# Autodesk Inventor assembly: Drivebase
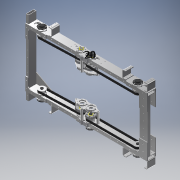
[picture p0: Inventor's stored thumbnail of the model, 180x180]
Saved by Autodesk Inventor 2019.4 (Build 234330000, 330)
## iProperties
Created: 2020-01-05
Part Number: Drivebase
Document SubType Name: Assembly
Designer: Mark
Mass: 11947.6 g
Surface Area: 25724.3 cm^2
Volume: 4557.12 cm^3
Density: 2.62175 g/cm^3
Author: Mark
## Documents named in this file (32)
- C:\Users\Mark\Desktop\7738 Helion Engineering\7738-2020\CAD\Drivebase.iam
- C:\Users\Mark\Desktop\7738 Helion Engineering\7738-2020\CAD\Main Extrusion.ipt
- C:\Users\Mark\Desktop\7738 Helion Engineering\7738-2020\CAD\Back Extrusion.ipt
- C:\Users\Mark\Desktop\7738 Helion Engineering\7738-2020\CAD\Bearing Block Assembly.iam
- C:\Users\Mark\Desktop\7738 Helion Engineering\7738-2020\CAD\Gearbox\Drivebox.iam
- C:\Users\Mark\Desktop\7738 Helion Engineering\7738-2020\CAD\End Extrusion.ipt
- C:\Users\Mark\Desktop\7738 Helion Engineering\7738-2020\CAD\Gearbox\HTD 5M 30 20mm ID Keyed.ipt
- C:\Users\Mark\Desktop\7738 Helion Engineering\7738-2020\CAD\Gearbox\30-30-870-HTD5M.ipt
- C:\Users\Mark\Desktop\7738 Helion Engineering\7738-2020\CAD\Gearbox\30-30-750-HTD5M.ipt
- C:\Users\Mark\Desktop\7738 Helion Engineering\7738-2020\CAD\Frontal Sheet Metal Support.ipt
- C:\Users\Mark\Desktop\7738 Helion Engineering\7738-2020\CAD\Shaft-Secondary.ipt
- C:\Users\Mark\Desktop\7738 Helion Engineering\7738-2020\CAD\Drivebase\Design Accelerator\Key Connection1.iam
- C:\Users\Mark\Desktop\7738 Helion Engineering\7738-2020\CAD\Shaft-2.ipt
- C:\Users\Mark\Desktop\7738 Helion Engineering\7738-2020\CAD\Back Brace.ipt
- C:\Users\Mark\Desktop\7738 Helion Engineering\7738-2020\CAD\Back brace 2.ipt
- C:\Users\Mark\Desktop\7738 Helion Engineering\7738-2020\CAD\Front Brace 2.ipt
- C:\Users\Mark\Desktop\7738 Helion Engineering\7738-2020\CAD\Gearbox Support Thing.ipt
- C:\Users\Mark\Desktop\7738 Helion Engineering\7738-2020\CAD\Main Extrusion_MIR.ipt
- C:\Users\Mark\Desktop\7738 Helion Engineering\7738-2020\CAD\Bearing Block Assembly_MIR.iam
- C:\Users\Mark\Desktop\7738 Helion Engineering\7738-2020\CAD\Gearbox\Drivebox_MIR.iam
- C:\Users\Mark\Desktop\7738 Helion Engineering\7738-2020\CAD\Gearbox\HTD 5M 30 20mm ID Keyed_MIR.ipt
- C:\Users\Mark\Desktop\7738 Helion Engineering\7738-2020\CAD\Gearbox\30-30-870-HTD5M_MIR.ipt
- C:\Users\Mark\Desktop\7738 Helion Engineering\7738-2020\CAD\Gearbox\30-30-750-HTD5M_MIR.ipt
- C:\Users\Mark\Desktop\7738 Helion Engineering\7738-2020\CAD\Frontal Sheet Metal Support_MIR.ipt
- C:\Users\Mark\Desktop\7738 Helion Engineering\7738-2020\CAD\Shaft-Secondary_MIR.ipt
- C:\Users\Mark\Desktop\7738 Helion Engineering\7738-2020\CAD\Drivebase\Design Accelerator\Key Connection1_MIR.iam
- C:\Users\Mark\Desktop\7738 Helion Engineering\7738-2020\CAD\Shaft-Main_MIR.ipt
- C:\Users\Mark\Desktop\7738 Helion Engineering\7738-2020\CAD\Shaft-2_MIR.ipt
- C:\Users\Mark\Desktop\7738 Helion Engineering\7738-2020\CAD\Back Brace_MIR.ipt
- C:\Users\Mark\Desktop\7738 Helion Engineering\7738-2020\CAD\Back brace 2_MIR.ipt
- C:\Users\Mark\Desktop\7738 Helion Engineering\7738-2020\CAD\Gearbox Support Thing_MIR.ipt
- C:\Users\Mark\Desktop\7738 Helion Engineering\7738-2020\CAD\Shaft-Main.ipt
## Components (52 placed, 31 different names)
1. Main Extrusion:1 — Mate:1, Flush:1, Flush:2, Mate:2, Mate:3, Mate:4, Mate:5, Mate:6, Mate:7, Mate:8, Mate:9, Mate:10, Mate:11, Mate:12, Mate:13, Mate:14, Mate:15, Mate:16, Mate:17, Mate:18, Mate:19, Mate:27, Mate:30, Flush:3, Mate:31, Flush:4, Flush:5, Flush:6, Flush:7, Mate:42, Mate:43, Flush:8, Mate:49, Flush:11, Mate:61, Flush:14, Flush:15, Mate:63, Flush:18, Flush:19, Mate:64, Flush:20, Flush:21, Mate:65, Flush:22, Mate:124, Flush:43, Flush:44
2. Back Extrusion:1 — Mate:1, Flush:1, Flush:2, Mate:50, Mate:119, Flush:39, Flush:40
3. Bearing Block Assembly:1 [sub-assembly] — Mate:2, Mate:3, Mate:4, Mate:32, Mate:33
4. Bearing Block Assembly:2 [sub-assembly] — Mate:5, Mate:6, Mate:7, Mate:34, Mate:35
5. Bearing Block Assembly:3 [sub-assembly] — Mate:11, Mate:12, Mate:13, Mate:53, Mate:127
6. Bearing Block Assembly:4 [sub-assembly] — Mate:8, Mate:9, Mate:10, Mate:126
7. Bearing Block Assembly:5 [sub-assembly] — Mate:14, Mate:15, Mate:16, Mate:60, Flush:13
8. Bearing Block Assembly:6 [sub-assembly] — Mate:17, Mate:18, Mate:19, Mate:37, Mate:132, Mate:133
9. Drivebox:1 [sub-assembly] — Mate:27, Mate:31, Flush:4, Mate:40, Mate:121
10. End Extrusion:1 — Mate:30, Flush:3, Flush:5, Flush:46
11. HTD 5M 30 20mm ID Keyed:1 — Mate:32, Mate:33, Mate:39, Mate:41
12. HTD 5M 30 20mm ID Keyed:2 — Mate:34, Mate:35, Mate:36, Mate:38
13. 30-30-870-HTD5M:1 — Mate:36, Mate:37, Mate:38
14. 30-30-730-HTD5M:1 — Mate:39, Mate:40, Mate:41
15. Frontal Sheet Metal Support:1 — Flush:6, Flush:7, Mate:42, Mate:44
16. Frontal Sheet Metal Support:2 — Mate:43, Flush:8, Mate:44
17. Frontal Sheet Metal Support:5 — Mate:49, Flush:11, Mate:50
18. Shaft-Secondary:1 — Mate:53, Mate:127
19. Shaft-Secondary:2 — Mate:126
20. Key Connection:1 [sub-assembly]
21. Shaft-2:1 — Mate:60, Flush:13
22. Back Brace:1 — Mate:61, Flush:14, Flush:15
23. Back brace 2:1 — Mate:63, Flush:18, Flush:19
24. Front Brace 2:1 — Mate:64, Flush:20, Flush:21
25. Gearbox Support Thing:1 — Mate:65, Flush:22, Mate:121
26. Main Extrusion_MIR:1 — Mate:66, Mate:67, Mate:68, Mate:69, Mate:70, Mate:71, Mate:72, Mate:73, Mate:74, Mate:75, Mate:76, Mate:77, Mate:78, Mate:79, Mate:80, Mate:81, Mate:82, Mate:83, Flush:23, Mate:89, Mate:90, Mate:101, Flush:24, Flush:25, Flush:26, Mate:103, Flush:27, Mate:104, Flush:30, Flush:31, Mate:114, Flush:34, Flush:35, Mate:116, Flush:38, Mate:118, Mate:119, Flush:39, Flush:40, Mate:122, Mate:123, Flush:41, Flush:42, Mate:125, Flush:45
27. Bearing Block Assembly_MIR:1 [sub-assembly] — Mate:66, Mate:67, Mate:68, Mate:91, Mate:92
28. Bearing Block Assembly_MIR:2 [sub-assembly] — Mate:69, Mate:70, Mate:71, Mate:93, Mate:94
29. Bearing Block Assembly_MIR:3 [sub-assembly] — Mate:72, Mate:73, Mate:74, Mate:107, Mate:129
30. Bearing Block Assembly_MIR:4 [sub-assembly] — Mate:75, Mate:76, Mate:77, Mate:128, Mate:130
31. Bearing Block Assembly_MIR:5 [sub-assembly] — Mate:78, Mate:79, Mate:80, Flush:29, Mate:113
32. Bearing Block Assembly_MIR:6 [sub-assembly] — Mate:81, Mate:82, Mate:83, Mate:96, Mate:110
33. Drivebox_MIR:1 [sub-assembly] — Flush:23, Mate:89, Mate:90, Mate:99, Mate:131
34. HTD 5M 30 20mm ID Keyed_MIR:1 — Mate:91, Mate:92, Mate:98, Mate:100
35. HTD 5M 30 20mm ID Keyed_MIR:2 — Mate:93, Mate:94, Mate:95, Mate:97
36. 30-30-870-HTD5M_MIR:1 — Mate:95, Mate:96, Mate:97
37. 30-30-730-HTD5M_MIR:1 — Mate:98, Mate:99, Mate:100
38. Frontal Sheet Metal Support_MIR:1 — Mate:101, Flush:24, Flush:25, Mate:102
39. Frontal Sheet Metal Support_MIR:2 — Mate:102, Flush:26, Mate:103
40. Frontal Sheet Metal Support_MIR:3 — Flush:27, Mate:104, Mate:122
41. Shaft-Secondary_MIR:1 — Mate:107, Mate:129
42. Shaft-Secondary_MIR:2 — Mate:128, Mate:130
43. Key Connection1_MIR:1 [sub-assembly]
44. Shaft-Main_MIR:1 — Mate:110
45. Shaft-2_MIR:1 — Flush:29, Mate:113
46. Back Brace_MIR:1 — Flush:30, Flush:31, Mate:114
47. Back brace 2_MIR:1 — Flush:34, Flush:35, Mate:116
48. Gearbox Support Thing_MIR:1 — Flush:38, Mate:118, Mate:131
49. Front Brace 2:2 — Mate:123, Flush:41, Flush:42
50. Front Brace 2:3 — Mate:124, Flush:43, Flush:44
51. Front Brace 2:4 — Mate:125, Flush:45, Flush:46
52. Shaft-Main:1 — Mate:132, Mate:133
## Relationships (133: Mate 97, Flush 36)
- Mate:1: Main Extrusion:1 ↔ Back Extrusion:1
- Flush:1: Main Extrusion:1 ↔ Back Extrusion:1
- Flush:2 (-60 mm): Main Extrusion:1 ↔ Back Extrusion:1
- Mate:2: Main Extrusion:1 ↔ Bearing Block Assembly:1
- Mate:3: Main Extrusion:1 ↔ Bearing Block Assembly:1
- Mate:4: Main Extrusion:1 ↔ Bearing Block Assembly:1
- Mate:5: Main Extrusion:1 ↔ Bearing Block Assembly:2
- Mate:6: Main Extrusion:1 ↔ Bearing Block Assembly:2
- Mate:7: Main Extrusion:1 ↔ Bearing Block Assembly:2
- Mate:8: Main Extrusion:1 ↔ Bearing Block Assembly:4
- Mate:9: Main Extrusion:1 ↔ Bearing Block Assembly:4
- Mate:10: Main Extrusion:1 ↔ Bearing Block Assembly:4
- Mate:11: Main Extrusion:1 ↔ Bearing Block Assembly:3
- Mate:12: Main Extrusion:1 ↔ Bearing Block Assembly:3
- Mate:13: Main Extrusion:1 ↔ Bearing Block Assembly:3
- Mate:14: Main Extrusion:1 ↔ Bearing Block Assembly:5
- Mate:15: Main Extrusion:1 ↔ Bearing Block Assembly:5
- Mate:16: Main Extrusion:1 ↔ Bearing Block Assembly:5
- Mate:17: Main Extrusion:1 ↔ Bearing Block Assembly:6
- Mate:18: Main Extrusion:1 ↔ Bearing Block Assembly:6
- Mate:19: Main Extrusion:1 ↔ Bearing Block Assembly:6
- Mate:27: Main Extrusion:1 ↔ Drivebox:1
- Mate:30: Main Extrusion:1 ↔ End Extrusion:1
- Flush:3: Main Extrusion:1 ↔ End Extrusion:1
- Mate:31: Main Extrusion:1 ↔ Drivebox:1
- Flush:4: Main Extrusion:1 ↔ Drivebox:1
- Mate:32: Bearing Block Assembly:1 ↔ HTD 5M 30 20mm ID Keyed:1
- Mate:33 (3 mm): Bearing Block Assembly:1 ↔ HTD 5M 30 20mm ID Keyed:1
- Flush:5: Main Extrusion:1 ↔ End Extrusion:1
- Mate:34: Bearing Block Assembly:2 ↔ HTD 5M 30 20mm ID Keyed:2
- Mate:35 (3 mm): Bearing Block Assembly:2 ↔ HTD 5M 30 20mm ID Keyed:2
- Mate:36: HTD 5M 30 20mm ID Keyed:2 ↔ 30-30-870-HTD5M:1
- Mate:37: Bearing Block Assembly:6 ↔ 30-30-870-HTD5M:1
- Mate:38 (0.5 mm): HTD 5M 30 20mm ID Keyed:2 ↔ 30-30-870-HTD5M:1
- Mate:39: HTD 5M 30 20mm ID Keyed:1 ↔ 30-30-730-HTD5M:1
- Mate:40: Drivebox:1 ↔ 30-30-730-HTD5M:1
- Mate:41 (0.5 mm): HTD 5M 30 20mm ID Keyed:1 ↔ 30-30-730-HTD5M:1
- Flush:6: Main Extrusion:1 ↔ Frontal Sheet Metal Support:1
- Flush:7: Main Extrusion:1 ↔ Frontal Sheet Metal Support:1
- Mate:42: Main Extrusion:1 ↔ Frontal Sheet Metal Support:1
- Mate:43: Main Extrusion:1 ↔ Frontal Sheet Metal Support:2
- Flush:8: Main Extrusion:1 ↔ Frontal Sheet Metal Support:2
- Mate:44 (143 mm): Frontal Sheet Metal Support:1 ↔ Frontal Sheet Metal Support:2
- Mate:49: Main Extrusion:1 ↔ Frontal Sheet Metal Support:5
- Flush:11: Main Extrusion:1 ↔ Frontal Sheet Metal Support:5
- Mate:50 (173 mm): Back Extrusion:1 ↔ Frontal Sheet Metal Support:5
- Mate:53: Bearing Block Assembly:3 ↔ Shaft-Secondary:1
- Mate:60: Bearing Block Assembly:5 ↔ Shaft-2:1
- Flush:13 (-0.2 mm): Bearing Block Assembly:5 ↔ Shaft-2:1
- Mate:61: Main Extrusion:1 ↔ Back Brace:1
- Flush:14: Main Extrusion:1 ↔ Back Brace:1
- Flush:15 (-20 mm): Main Extrusion:1 ↔ Back Brace:1
- Mate:63: Main Extrusion:1 ↔ Back brace 2:1
- Flush:18: Main Extrusion:1 ↔ Back brace 2:1
- Flush:19 (-20 mm): Main Extrusion:1 ↔ Back brace 2:1
- Mate:64: Main Extrusion:1 ↔ Front Brace 2:1
- Flush:20: Main Extrusion:1 ↔ Front Brace 2:1
- Flush:21: Main Extrusion:1 ↔ Front Brace 2:1
- Mate:65: Main Extrusion:1 ↔ Gearbox Support Thing:1
- Flush:22: Main Extrusion:1 ↔ Gearbox Support Thing:1
- Mate:66: Main Extrusion_MIR:1 ↔ Bearing Block Assembly_MIR:1
- Mate:67: Main Extrusion_MIR:1 ↔ Bearing Block Assembly_MIR:1
- Mate:68: Main Extrusion_MIR:1 ↔ Bearing Block Assembly_MIR:1
- Mate:69: Main Extrusion_MIR:1 ↔ Bearing Block Assembly_MIR:2
- Mate:70: Main Extrusion_MIR:1 ↔ Bearing Block Assembly_MIR:2
- Mate:71: Main Extrusion_MIR:1 ↔ Bearing Block Assembly_MIR:2
- Mate:72: Main Extrusion_MIR:1 ↔ Bearing Block Assembly_MIR:3
- Mate:73: Main Extrusion_MIR:1 ↔ Bearing Block Assembly_MIR:3
- Mate:74: Main Extrusion_MIR:1 ↔ Bearing Block Assembly_MIR:3
- Mate:75: Main Extrusion_MIR:1 ↔ Bearing Block Assembly_MIR:4
- Mate:76: Main Extrusion_MIR:1 ↔ Bearing Block Assembly_MIR:4
- Mate:77: Main Extrusion_MIR:1 ↔ Bearing Block Assembly_MIR:4
- Mate:78: Main Extrusion_MIR:1 ↔ Bearing Block Assembly_MIR:5
- Mate:79: Main Extrusion_MIR:1 ↔ Bearing Block Assembly_MIR:5
- Mate:80: Main Extrusion_MIR:1 ↔ Bearing Block Assembly_MIR:5
- Mate:81: Main Extrusion_MIR:1 ↔ Bearing Block Assembly_MIR:6
- Mate:82: Main Extrusion_MIR:1 ↔ Bearing Block Assembly_MIR:6
- Mate:83: Main Extrusion_MIR:1 ↔ Bearing Block Assembly_MIR:6
- Flush:23: Main Extrusion_MIR:1 ↔ Drivebox_MIR:1
- Mate:89: Main Extrusion_MIR:1 ↔ Drivebox_MIR:1
- Mate:90: Main Extrusion_MIR:1 ↔ Drivebox_MIR:1
- Mate:91 (3 mm): Bearing Block Assembly_MIR:1 ↔ HTD 5M 30 20mm ID Keyed_MIR:1
- Mate:92: Bearing Block Assembly_MIR:1 ↔ HTD 5M 30 20mm ID Keyed_MIR:1
- Mate:93 (3 mm): Bearing Block Assembly_MIR:2 ↔ HTD 5M 30 20mm ID Keyed_MIR:2
- Mate:94: Bearing Block Assembly_MIR:2 ↔ HTD 5M 30 20mm ID Keyed_MIR:2
- Mate:95 (0.5 mm): HTD 5M 30 20mm ID Keyed_MIR:2 ↔ 30-30-870-HTD5M_MIR:1
- Mate:96: Bearing Block Assembly_MIR:6 ↔ 30-30-870-HTD5M_MIR:1
- Mate:97: HTD 5M 30 20mm ID Keyed_MIR:2 ↔ 30-30-870-HTD5M_MIR:1
- Mate:98 (0.5 mm): HTD 5M 30 20mm ID Keyed_MIR:1 ↔ 30-30-730-HTD5M_MIR:1
- Mate:99: Drivebox_MIR:1 ↔ 30-30-730-HTD5M_MIR:1
- Mate:100: HTD 5M 30 20mm ID Keyed_MIR:1 ↔ 30-30-730-HTD5M_MIR:1
- Mate:101: Main Extrusion_MIR:1 ↔ Frontal Sheet Metal Support_MIR:1
- Flush:24: Main Extrusion_MIR:1 ↔ Frontal Sheet Metal Support_MIR:1
- Flush:25: Main Extrusion_MIR:1 ↔ Frontal Sheet Metal Support_MIR:1
- Mate:102 (140 mm): Frontal Sheet Metal Support_MIR:1 ↔ Frontal Sheet Metal Support_MIR:2
- Flush:26: Main Extrusion_MIR:1 ↔ Frontal Sheet Metal Support_MIR:2
- Mate:103: Main Extrusion_MIR:1 ↔ Frontal Sheet Metal Support_MIR:2
- Flush:27: Main Extrusion_MIR:1 ↔ Frontal Sheet Metal Support_MIR:3
- Mate:104: Main Extrusion_MIR:1 ↔ Frontal Sheet Metal Support_MIR:3
- Mate:107: Bearing Block Assembly_MIR:3 ↔ Shaft-Secondary_MIR:1
- Mate:110 (6 mm): Bearing Block Assembly_MIR:6 ↔ Shaft-Main_MIR:1
- Flush:29 (-0.2 mm): Bearing Block Assembly_MIR:5 ↔ Shaft-2_MIR:1
- Mate:113: Bearing Block Assembly_MIR:5 ↔ Shaft-2_MIR:1
- Flush:30 (-20 mm): Main Extrusion_MIR:1 ↔ Back Brace_MIR:1
- Flush:31: Main Extrusion_MIR:1 ↔ Back Brace_MIR:1
- Mate:114: Main Extrusion_MIR:1 ↔ Back Brace_MIR:1
- Flush:34 (-20 mm): Main Extrusion_MIR:1 ↔ Back brace 2_MIR:1
- Flush:35: Main Extrusion_MIR:1 ↔ Back brace 2_MIR:1
- Mate:116: Main Extrusion_MIR:1 ↔ Back brace 2_MIR:1
- Flush:38: Main Extrusion_MIR:1 ↔ Gearbox Support Thing_MIR:1
- Mate:118: Main Extrusion_MIR:1 ↔ Gearbox Support Thing_MIR:1
- Mate:119: Back Extrusion:1 ↔ Main Extrusion_MIR:1
- Flush:39: Back Extrusion:1 ↔ Main Extrusion_MIR:1
- Flush:40 (60 mm): Back Extrusion:1 ↔ Main Extrusion_MIR:1
- Mate:121: Drivebox:1 ↔ Gearbox Support Thing:1
- Mate:122: Main Extrusion_MIR:1 ↔ Frontal Sheet Metal Support_MIR:3
- Mate:123: Main Extrusion_MIR:1 ↔ Front Brace 2:2
- Flush:41: Main Extrusion_MIR:1 ↔ Front Brace 2:2
- Flush:42: Main Extrusion_MIR:1 ↔ Front Brace 2:2
- Mate:124: Main Extrusion:1 ↔ Front Brace 2:3
- Flush:43: Main Extrusion:1 ↔ Front Brace 2:3
- Flush:44: Main Extrusion:1 ↔ Front Brace 2:3
- Mate:125: Main Extrusion_MIR:1 ↔ Front Brace 2:4
- Flush:45: Main Extrusion_MIR:1 ↔ Front Brace 2:4
- Flush:46: End Extrusion:1 ↔ Front Brace 2:4
- Mate:126 (6 mm): Bearing Block Assembly:4 ↔ Shaft-Secondary:2
- Mate:127 (6 mm): Bearing Block Assembly:3 ↔ Shaft-Secondary:1
- Mate:128 (6 mm): Bearing Block Assembly_MIR:4 ↔ Shaft-Secondary_MIR:2
- Mate:129 (6 mm): Bearing Block Assembly_MIR:3 ↔ Shaft-Secondary_MIR:1
- Mate:130: Bearing Block Assembly_MIR:4 ↔ Shaft-Secondary_MIR:2
- Mate:131: Drivebox_MIR:1 ↔ Gearbox Support Thing_MIR:1
- Mate:132: Bearing Block Assembly:6 ↔ Shaft-Main:1
- Mate:133 (6 mm): Bearing Block Assembly:6 ↔ Shaft-Main:1
